# Autodesk Inventor assembly: wadah_jerrycan
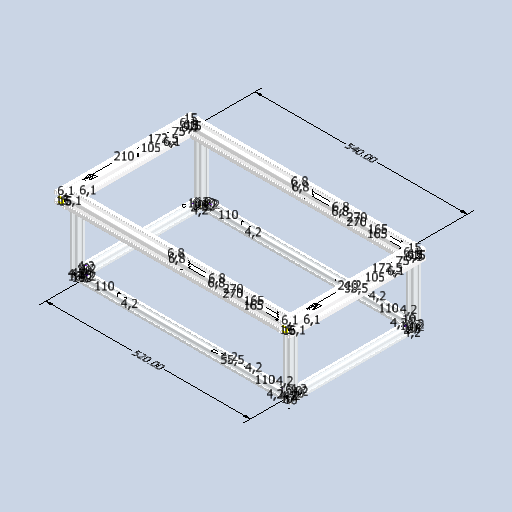
[picture p0: Inventor's stored thumbnail of the model, 512x512]
Saved by Autodesk Inventor 2023 (Build 270158000, 158)
## iProperties
Created: 2023-10-09
Part Number: wadah_jerrycan
Document SubType Name: Assembly
Designer: sigit
Author: sigit
## Documents named in this file (6)
- D:\Kuliah\SEMESTER 7\Robot Semprot\Design\2nd ROBOT\Assembly\wadah_jerrycan.iam
- D:\Kuliah\SEMESTER 7\Robot Semprot\Design\2nd ROBOT\Part\2020 295.ipt
- D:\Kuliah\SEMESTER 7\Robot Semprot\Design\2nd ROBOT\Part\2020 150.ipt
- D:\Kuliah\SEMESTER 7\Robot Semprot\Design\2nd ROBOT\Part\2020 520.ipt
- D:\Kuliah\SEMESTER 7\Robot Semprot\Design\2nd ROBOT\Part\3030 345.ipt
- D:\Kuliah\SEMESTER 7\Robot Semprot\Design\2nd ROBOT\Part\3030 540.ipt
## Components (12 placed, 5 different names)
1. 2020 520:1 — Rotational:2
2. 2020 520:2
3. 2020 295:1 — Rotational:1
4. 2020 295:2
5. 3030 540:1 — Rotational:4
6. 3030 540:2
7. 3030 345:1 — Rotational:3, Rotational:4
8. 3030 345:2
9. 2020 150:1 — Rotational:1, Rotational:2
10. 2020 150:2
11. 2020 150:3 — Rotational:3
12. 2020 150:4
## Component patterns: (2 elements, first: 2020 520:1), (2 elements, first: 2020 295:1), (2 elements, first: 3030 540:1), (2 elements, first: 3030 345:1), (2 elements, first: 2020 150:1), Component Pattern 1:2 (2 elements)
## Relationships (4: RevoluteJoint 4)
- Rotational:1 [RevoluteJoint] (6.1 mm): 2020 295:1 ↔ 2020 150:1
- Rotational:2 [RevoluteJoint] (6.1 mm): 2020 520:1 ↔ 2020 150:1
- Rotational:3 [RevoluteJoint] (-9.486 mm): 3030 345:1 ↔ 2020 150:3
- Rotational:4 [RevoluteJoint] (9.486 mm): 3030 540:1 ↔ 3030 345:1
